# Autodesk Inventor assembly: HEAD
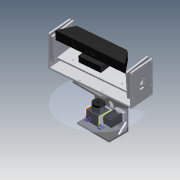
[picture p0: Inventor's stored thumbnail of the model, 180x180]
Saved by Autodesk Inventor 2011 (Build 150239000, 239)
## iProperties
Created: 2011-12-04
Part Number: HEAD
Document SubType Name: Assembly
Designer: Matthew
Author: Matthew
## Documents named in this file (21)
- C:\Users\Matthew\Documents\matthew_autocad\prlite\head\HEAD.iam
- C:\Users\Matthew\Documents\matthew_autocad\prlite\head\hokoyo\h base.ipt
- C:\Users\Matthew\Documents\matthew_autocad\prlite\head\hokoyo\hmodel.ipt
- C:\Users\Matthew\Documents\matthew_autocad\prlite\head\hokoyo\view2.ipt
- C:\Users\Matthew\Documents\matthew_autocad\prlite\head\hokoyo\sidebase.ipt
- C:\Users\Matthew\Documents\matthew_autocad\prlite\Bioloid\base1.ipt
- C:\Users\Matthew\Documents\matthew_autocad\prlite\head\hconnector.ipt
- C:\Users\Matthew\Documents\matthew_autocad\prlite\head\hconnector2.ipt
- C:\Users\Matthew\Documents\matthew_autocad\prlite\head\frontbase.ipt
- C:\Users\Matthew\Documents\matthew_autocad\prlite\head\bottombase.ipt
- C:\Users\Matthew\Documents\matthew_autocad\prlite\head\corner brace.ipt
- C:\Users\Matthew\Documents\matthew_autocad\prlite\head\kinect base closer holes.ipt
- C:\Users\Matthew\Documents\matthew_autocad\prlite\lazy susan\1.ipt
- C:\Users\Matthew\Documents\matthew_autocad\prlite\lazy susan\2.ipt
- C:\Users\Matthew\Documents\matthew_autocad\prlite\AX12\awesomebody.ipt
- C:\Users\Matthew\Documents\matthew_autocad\prlite\AX12\awesomespin.ipt
- C:\Users\Matthew\Documents\matthew_autocad\prlite\head\kinect rotate bottom.ipt
- C:\Users\Matthew\Documents\matthew_autocad\prlite\other\kinect basic.ipt
- C:\Users\Matthew\Documents\matthew_autocad\prlite\head\kinect rotate side.ipt
- C:\Users\Matthew\Documents\matthew_autocad\prlite\head\kinect rotate2 side.ipt
- C:\Users\Matthew\Documents\matthew_autocad\prlite\head\kinect rotate2 bottom.ipt
## Components (27 placed, 20 different names)
1. h base:1 — Mate:1, Mate:2, Mate:3, Flush:2, Mate:79, Flush:43, Flush:45
2. hmodel:1 — Mate:1, Mate:2, Mate:3, Mate:4, Mate:5, Mate:6
3. view2:1 — Mate:4, Mate:5, Mate:6
4. sidebase:1 — Flush:2, Mate:44, Mate:45, Mate:46, Mate:79, Flush:43, Flush:45
5. base1:1 — Flush:10, Flush:11, Mate:49, Flush:22, Mate:80, Flush:44
6. hconnector:1 — Flush:10, Flush:11, Mate:23, Mate:77, Mate:78, Mate:80
7. hconnector2:1 — Mate:75, Mate:76, Flush:42
8. frontbase:1 — Mate:23, Flush:13, Mate:25, Mate:32, Mate:35, Flush:21, Mate:38, Flush:38, Flush:39, Flush:40, Flush:41, Mate:75, Mate:76, Mate:77, Mate:78, Flush:42
9. bottombase:1 — Flush:13, Mate:25, Flush:38
10. corner brace:3 — Mate:32, Mate:37, Flush:41
11. corner brace:4 — Mate:35, Mate:36, Flush:40
12. kinect base closer holes:1 — Flush:21, Mate:36, Mate:37, Mate:38, Mate:39, Mate:40, Mate:41, Flush:39, Flush:46
13. 1:1 — Mate:42, Mate:43, Mate:50, Mate:51, Mate:52, Angle:1
14. 2:1 — Mate:39, Mate:40, Mate:41, Mate:42, Mate:43, Angle:1
15. awesomebody:1 — Mate:47, Mate:48, Mate:49, Flush:22, Flush:44
16. awesomespin:1 — Mate:44, Mate:45, Mate:46, Mate:47, Mate:48
17. kinect rotate bottom:1 — Mate:50, Mate:51, Mate:52, Flush:24, Flush:25, Flush:27, Flush:28, HEIGHT, Flush:46
18. kinect basic:1 — Mate:73, Flush:35, Flush:37
19. kinect rotate side:1 — Flush:24, Flush:25, Flush:26, HEIGHT, Mate:59, Mate:60, Mate:61
20. kinect rotate side:2 — Flush:26, Flush:27, Flush:28, Mate:58, Mate:62, Mate:63
21. 1:2 — Mate:54, Mate:55, Mate:59, Mate:60, Mate:61
22. 1:3 — Mate:56, Mate:57, Mate:58, Mate:62, Mate:63
23. 2:2 — Mate:56, Mate:57, Flush:30, Mate:64, Mate:68, Mate:69
24. 2:3 — Mate:54, Mate:55, Flush:30, Mate:70, Mate:71, Mate:72
25. kinect rotate2 side:1 — Mate:64, Mate:68, Mate:69, Flush:32, Flush:36, Flush:37, Mate:74
26. kinect rotate2 bottom:1 — Flush:32, Flush:36, Mate:74
27. kinect rotate2 side:2 — Mate:70, Mate:71, Mate:72, Mate:73, Flush:35
## Relationships (78: Mate 51, Flush 26, Angle 1)
- Mate:1: h base:1 ↔ hmodel:1
- Mate:2: h base:1 ↔ hmodel:1
- Mate:3: h base:1 ↔ hmodel:1
- Mate:4: hmodel:1 ↔ view2:1
- Mate:5: hmodel:1 ↔ view2:1
- Mate:6: hmodel:1 ↔ view2:1
- Flush:2: h base:1 ↔ sidebase:1
- Flush:10: base1:1 ↔ hconnector:1
- Flush:11: base1:1 ↔ hconnector:1
- Mate:23: hconnector:1 ↔ frontbase:1
- Flush:13: frontbase:1 ↔ bottombase:1
- Mate:25: frontbase:1 ↔ bottombase:1
- Mate:32: frontbase:1 ↔ corner brace:3
- Mate:35: frontbase:1 ↔ corner brace:4
- Flush:21: frontbase:1 ↔ kinect base closer holes:1
- Mate:36: corner brace:4 ↔ kinect base closer holes:1
- Mate:37: corner brace:3 ↔ kinect base closer holes:1
- Mate:38: frontbase:1 ↔ kinect base closer holes:1
- Mate:39: kinect base closer holes:1 ↔ 2:1
- Mate:40: kinect base closer holes:1 ↔ 2:1
- Mate:41: kinect base closer holes:1 ↔ 2:1
- Mate:42: 1:1 ↔ 2:1
- Mate:43: 1:1 ↔ 2:1
- Mate:44: sidebase:1 ↔ awesomespin:1
- Mate:45: sidebase:1 ↔ awesomespin:1
- Mate:46: sidebase:1 ↔ awesomespin:1
- Mate:47: awesomebody:1 ↔ awesomespin:1
- Mate:48: awesomebody:1 ↔ awesomespin:1
- Mate:49: base1:1 ↔ awesomebody:1
- Flush:22: base1:1 ↔ awesomebody:1
- Mate:50: 1:1 ↔ kinect rotate bottom:1
- Mate:51: 1:1 ↔ kinect rotate bottom:1
- Mate:52: 1:1 ↔ kinect rotate bottom:1
- Angle:1 (0 deg): 1:1 ↔ 2:1
- Flush:24: kinect rotate bottom:1 ↔ kinect rotate side:1
- Flush:25: kinect rotate bottom:1 ↔ kinect rotate side:1
- Flush:26: kinect rotate side:1 ↔ kinect rotate side:2
- Flush:27: kinect rotate bottom:1 ↔ kinect rotate side:2
- Flush:28: kinect rotate bottom:1 ↔ kinect rotate side:2
- HEIGHT [Flush] (-127 mm): kinect rotate bottom:1 ↔ kinect rotate side:1
- Mate:54: 1:2 ↔ 2:3
- Mate:55: 1:2 ↔ 2:3
- Mate:56: 1:3 ↔ 2:2
- Mate:57: 1:3 ↔ 2:2
- Mate:58: kinect rotate side:2 ↔ 1:3
- Mate:59: kinect rotate side:1 ↔ 1:2
- Mate:60: kinect rotate side:1 ↔ 1:2
- Mate:61: kinect rotate side:1 ↔ 1:2
- Mate:62: kinect rotate side:2 ↔ 1:3
- Mate:63: kinect rotate side:2 ↔ 1:3
- Flush:30: 2:2 ↔ 2:3
- Mate:64: 2:2 ↔ kinect rotate2 side:1
- Mate:68: 2:2 ↔ kinect rotate2 side:1
- Mate:69: 2:2 ↔ kinect rotate2 side:1
- Flush:32 (5.334 mm): kinect rotate2 side:1 ↔ kinect rotate2 bottom:1
- Mate:70: 2:3 ↔ kinect rotate2 side:2
- Mate:71: 2:3 ↔ kinect rotate2 side:2
- Mate:72: 2:3 ↔ kinect rotate2 side:2
- Mate:73 (101.6 mm): kinect basic:1 ↔ kinect rotate2 side:2
- Flush:35 (50.546 mm): kinect basic:1 ↔ kinect rotate2 side:2
- Flush:36: kinect rotate2 side:1 ↔ kinect rotate2 bottom:1
- Flush:37: kinect basic:1 ↔ kinect rotate2 side:1
- Mate:74 (0.762 mm): kinect rotate2 side:1 ↔ kinect rotate2 bottom:1
- Flush:38: frontbase:1 ↔ bottombase:1
- Flush:39: frontbase:1 ↔ kinect base closer holes:1
- Flush:40: frontbase:1 ↔ corner brace:4
- Flush:41: frontbase:1 ↔ corner brace:3
- Mate:75: hconnector2:1 ↔ frontbase:1
- Mate:76: hconnector2:1 ↔ frontbase:1
- Mate:77: hconnector:1 ↔ frontbase:1
- Mate:78: hconnector:1 ↔ frontbase:1
- Flush:42: hconnector2:1 ↔ frontbase:1
- Mate:79: h base:1 ↔ sidebase:1
- Mate:80: base1:1 ↔ hconnector:1
- Flush:43: h base:1 ↔ sidebase:1
- Flush:44 (1 mm): base1:1 ↔ awesomebody:1
- Flush:45: h base:1 ↔ sidebase:1
- Flush:46: kinect base closer holes:1 ↔ kinect rotate bottom:1
